# Autodesk Inventor assembly: HS Conveyor Axle
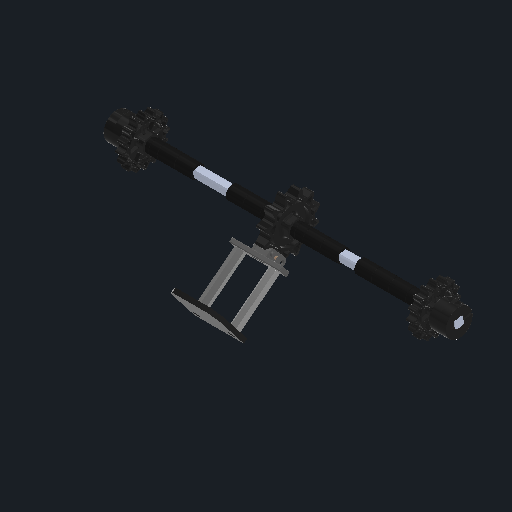
[picture p0: Inventor's stored thumbnail of the model, 512x512]
Saved by Autodesk Inventor 2025 (Build 290162000, 162)
## iProperties
Created: 2024-12-19
Part Number: HS Conveyor Axle
Document SubType Name: Assembly
Designer: Juan
Author: Juan
## Documents named in this file (16)
- C:\Users\Juan\Documents\GitHub\ATUM-VRC-High-Stakes-CAD\Protobot\HS Conveyor Axle.iam
- C:\Users\Juan\Documents\GitHub\ATUM-VRC-High-Stakes-CAD\VEX-CAD-Inventor\Motion\Shaft HS\Shaft HS\Shaft HS 10.0 in.ipt
- C:\Users\Juan\Documents\GitHub\ATUM-VRC-High-Stakes-CAD\VEX-CAD-Inventor\Motion\Shaft HS\Shaft HS.ipt
- C:\Users\Juan\Documents\GitHub\ATUM-VRC-High-Stakes-CAD\VEX-CAD-Inventor\Motion\Shaft HS\HS Spacer\HSpacer .5000.ipt
- C:\Users\Juan\Documents\GitHub\ATUM-VRC-High-Stakes-CAD\VEX-CAD-Inventor\Motion\Shaft HS\HS Spacer.ipt
- C:\Users\Juan\Documents\GitHub\ATUM-VRC-High-Stakes-CAD\VEX-CAD-Inventor\Motion\Shaft HS\HS Spacer\HSpacer .2500.ipt
- C:\Users\Juan\Documents\GitHub\ATUM-VRC-High-Stakes-CAD\VEX-CAD-Inventor\Motion\Shaft HS\HS Spacer\HSpacer .1250.ipt
- C:\Users\Juan\Documents\GitHub\ATUM-VRC-High-Stakes-CAD\VEX-CAD-Inventor\Motion\Sprockets\9P Sprocket\9P 12T Sprocket, Circle.iam
- C:\Users\Juan\Documents\GitHub\ATUM-VRC-High-Stakes-CAD\VEX-CAD-Inventor\Motion\Sprockets\9P Sprocket.iam
- C:\Users\Juan\Documents\GitHub\ATUM-VRC-High-Stakes-CAD\VEX-CAD-Inventor\Motion\Sprockets\6P Sprocket\6P 16T Sprocket, No Insert.iam
- C:\Users\Juan\Documents\GitHub\ATUM-VRC-High-Stakes-CAD\VEX-CAD-Inventor\Motion\Sprockets\6P Sprocket.iam
- C:\Users\Juan\Documents\GitHub\ATUM-VRC-High-Stakes-CAD\VEX-CAD-Inventor\Motion\Shaft HS\HS Shaft Collar.ipt
- C:\Users\Juan\Documents\GitHub\ATUM-VRC-High-Stakes-CAD\VEX-CAD-Inventor\Motion\Chain 9P\Chain Attachment Link.ipt
- C:\Users\Juan\Documents\GitHub\ATUM-VRC-High-Stakes-CAD\Hook.ipt
- C:\Users\Juan\Documents\GitHub\ATUM-VRC-High-Stakes-CAD\VEX-CAD-Inventor\Structure\Standoff\Standoff 1.50.ipt
- C:\Users\Juan\Documents\GitHub\ATUM-VRC-High-Stakes-CAD\VEX-CAD-Inventor\Structure\Standoff.ipt
## Components (27 placed, 10 different names)
1. Shaft HS 10.0 in:1
2. HSpacer .5000:1
3. HSpacer .5000:2
4. HSpacer .5000:3
5. Chain Attachment Link:1
6. Standoff 1.50:2
7. Standoff 1.50:1
8. Hook:1
9. HSpacer .5000:4
10. HSpacer .5000:5
11. HSpacer .5000:6
12. HSpacer .5000:7
13. HSpacer .5000:8
14. HSpacer .5000:9
15. HSpacer .2500:10
16. HSpacer .2500:11
17. HSpacer .1250:12
18. HSpacer .1250:13
19. 9P 12T Sprocket, Circle:1 [sub-assembly]
20. HSpacer .2500:14
21. HSpacer .2500:15
22. HSpacer .1250:16
23. HSpacer .1250:17
24. 6P 16T Sprocket, No Insert:1 [sub-assembly]
25. 6P 16T Sprocket, No Insert:2 [sub-assembly]
26. HS Shaft Collar:1
27. HS Shaft Collar:2
## Relationships (72: Mate 72)
- [Mate]: Shaft HS 10.0 in:1 ↔ HSpacer .5000:1
- [Mate]: Shaft HS 10.0 in:1 ↔ HSpacer .5000:1
- [Mate]: Shaft HS 10.0 in:1 ↔ HSpacer .5000:2
- [Mate]: Shaft HS 10.0 in:1 ↔ HSpacer .5000:2
- [Mate]: Shaft HS 10.0 in:1 ↔ HSpacer .5000:4
- [Mate]: Shaft HS 10.0 in:1 ↔ HSpacer .5000:4
- [Mate]: Shaft HS 10.0 in:1 ↔ HSpacer .5000:3
- [Mate]: Shaft HS 10.0 in:1 ↔ HSpacer .5000:3
- [Mate]: Shaft HS 10.0 in:1 ↔ HSpacer .5000:6
- [Mate]: Shaft HS 10.0 in:1 ↔ HSpacer .5000:6
- [Mate]: Shaft HS 10.0 in:1 ↔ HSpacer .5000:7
- [Mate]: Shaft HS 10.0 in:1 ↔ HSpacer .5000:7
- [Mate]: Shaft HS 10.0 in:1 ↔ HSpacer .5000:5
- [Mate]: Shaft HS 10.0 in:1 ↔ HSpacer .5000:5
- [Mate]: Shaft HS 10.0 in:1 ↔ HSpacer .5000:9
- [Mate]: Shaft HS 10.0 in:1 ↔ HSpacer .5000:9
- [Mate]: Shaft HS 10.0 in:1 ↔ HSpacer .5000:8
- [Mate]: Shaft HS 10.0 in:1 ↔ HSpacer .5000:8
- [Mate]: HSpacer .5000:3 ↔ HSpacer .5000:5
- [Mate]: HSpacer .5000:5 ↔ HSpacer .5000:8
- [Mate]: HSpacer .5000:1 ↔ HSpacer .5000:2
- [Mate]: HSpacer .5000:6 ↔ HSpacer .5000:7
- [Mate]: HSpacer .5000:4 ↔ HSpacer .5000:9
- [Mate]: Shaft HS 10.0 in:1 ↔ HSpacer .2500:11
- [Mate]: Shaft HS 10.0 in:1 ↔ HSpacer .2500:11
- [Mate]: HSpacer .5000:9 ↔ HSpacer .2500:11
- [Mate]: Shaft HS 10.0 in:1 ↔ HSpacer .2500:10
- [Mate]: Shaft HS 10.0 in:1 ↔ HSpacer .2500:10
- [Mate]: HSpacer .5000:6 ↔ HSpacer .2500:10
- [Mate]: Shaft HS 10.0 in:1 ↔ HSpacer .1250:12
- [Mate]: Shaft HS 10.0 in:1 ↔ HSpacer .1250:12
- [Mate]: HSpacer .2500:11 ↔ HSpacer .1250:12
- [Mate]: Shaft HS 10.0 in:1 ↔ HSpacer .1250:13
- [Mate]: Shaft HS 10.0 in:1 ↔ HSpacer .1250:13
- [Mate]: HSpacer .2500:10 ↔ HSpacer .1250:13
- [Mate]: Shaft HS 10.0 in:1 ↔ 9P 12T Sprocket, Circle:1
- [Mate]: Shaft HS 10.0 in:1 ↔ 9P 12T Sprocket, Circle:1
- [Mate]: HSpacer .1250:12 ↔ 9P 12T Sprocket, Circle:1
- [Mate]: Shaft HS 10.0 in:1 ↔ HSpacer .2500:14
- [Mate]: Shaft HS 10.0 in:1 ↔ HSpacer .2500:14
- [Mate]: HSpacer .5000:8 ↔ HSpacer .2500:14
- [Mate]: Shaft HS 10.0 in:1 ↔ HSpacer .2500:15
- [Mate]: Shaft HS 10.0 in:1 ↔ HSpacer .2500:15
- [Mate]: HSpacer .5000:2 ↔ HSpacer .2500:15
- [Mate]: Shaft HS 10.0 in:1 ↔ HSpacer .1250:16
- [Mate]: Shaft HS 10.0 in:1 ↔ HSpacer .1250:16
- [Mate]: HSpacer .2500:14 ↔ HSpacer .1250:16
- [Mate]: Shaft HS 10.0 in:1 ↔ HSpacer .1250:17
- [Mate]: Shaft HS 10.0 in:1 ↔ HSpacer .1250:17
- [Mate]: HSpacer .2500:15 ↔ HSpacer .1250:17
- [Mate]: Shaft HS 10.0 in:1 ↔ 6P 16T Sprocket, No Insert:1
- [Mate]: Shaft HS 10.0 in:1 ↔ 6P 16T Sprocket, No Insert:1
- [Mate]: HSpacer .1250:16 ↔ 6P 16T Sprocket, No Insert:1
- [Mate]: Shaft HS 10.0 in:1 ↔ 6P 16T Sprocket, No Insert:2
- [Mate]: Shaft HS 10.0 in:1 ↔ 6P 16T Sprocket, No Insert:2
- [Mate]: HSpacer .1250:17 ↔ 6P 16T Sprocket, No Insert:2
- [Mate]: Shaft HS 10.0 in:1 ↔ HS Shaft Collar:1
- [Mate]: Shaft HS 10.0 in:1 ↔ HS Shaft Collar:1
- [Mate]: 6P 16T Sprocket, No Insert:1 ↔ HS Shaft Collar:1
- [Mate]: Shaft HS 10.0 in:1 ↔ HS Shaft Collar:2
- [Mate]: Shaft HS 10.0 in:1 ↔ HS Shaft Collar:2
- [Mate]: 6P 16T Sprocket, No Insert:2 ↔ HS Shaft Collar:2
- [Mate]: Chain Attachment Link:1 ↔ 9P 12T Sprocket, Circle:1
- [Mate] (-2.54 mm): Chain Attachment Link:1 ↔ 9P 12T Sprocket, Circle:1
- [Mate]: Chain Attachment Link:1 ↔ Standoff 1.50:1
- [Mate]: Chain Attachment Link:1 ↔ Standoff 1.50:2
- [Mate]: Chain Attachment Link:1 ↔ Standoff 1.50:2
- [Mate] (0.1524 mm): Chain Attachment Link:1 ↔ 9P 12T Sprocket, Circle:1
- [Mate]: Chain Attachment Link:1 ↔ Standoff 1.50:1
- [Mate]: Standoff 1.50:1 ↔ Hook:1
- [Mate]: Standoff 1.50:2 ↔ Hook:1
- [Mate]: Standoff 1.50:2 ↔ Hook:1
## Named parameters: d1464_d938 = 0 mm, d1465_d929 = 0 mm, d1466_d930 = -2.54 mm, d1467_d931 = 0 mm, d1468_d932 = 0 mm, d1469_d933 = 0 mm, d1470_d934 = 0.1524 mm, d1471_d935 = 0 mm, d1472_d936 = 0 mm, d1473_d937 = 0 mm
